# Autodesk Inventor assembly: intake
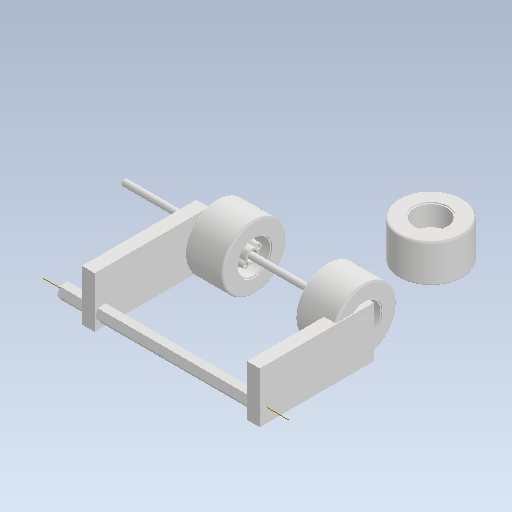
[picture p0: Inventor's stored thumbnail of the model, 512x512]
Saved by Autodesk Inventor 2021 (Build 250183000, 183)
## iProperties
Created: 2020-11-19
Part Number: intake
Document SubType Name: Assembly
Designer: gabe3
Author: gabe3
## Documents named in this file (5)
- C:\Robotics\CAD\2020-21-CAD\intake\intake.iam
- C:\Robotics\CAD\2020-21-CAD\intake\clolecton wheel holder.ipt
- C:\Robotics\CAD\2020-21-CAD\custom parts\.25 axle 9.5in.ipt
- C:\Robotics\CAD\COTSParts\Wheels\2.5inFoamWheel250TMD.ipt
- C:\Robotics\CAD\2020-21-CAD\custom parts\axles\2in hex 8in.ipt
## Components (7 placed, 4 different names)
1. clolecton wheel holder:1 — Flush:1, Flush:2, Mate:1, Mate:2
2. clolecton wheel holder:2 — Flush:1, Flush:2, Mate:1, Flush:3, Mate:6, Flush:4
3. .25 axle size template:1 — Mate:2, Flush:3, Mate:4, Mate:5
4. 2.5inFoamWheel250TMD:1 — Mate:4
5. 2.5inFoamWheel250TMD:2
6. 2.5inFoamWheel250TMD:3 — Mate:5
7. 2in hex 8in:1 — Mate:6, Flush:4
## Relationships (9: Mate 5, Flush 4)
- Flush:1: clolecton wheel holder:1 ↔ clolecton wheel holder:2
- Flush:2: clolecton wheel holder:1 ↔ clolecton wheel holder:2
- Mate:1 (152.4 mm): clolecton wheel holder:1 ↔ clolecton wheel holder:2
- Mate:2: clolecton wheel holder:1 ↔ .25 axle size template:1
- Flush:3: clolecton wheel holder:2 ↔ .25 axle size template:1
- Mate:4: .25 axle size template:1 ↔ 2.5inFoamWheel250TMD:1
- Mate:5: .25 axle size template:1 ↔ 2.5inFoamWheel250TMD:3
- Mate:6: clolecton wheel holder:2 ↔ 2in hex 8in:1
- Flush:4: clolecton wheel holder:2 ↔ 2in hex 8in:1
